# Autodesk Inventor assembly: Baugruppe_Christian_Test
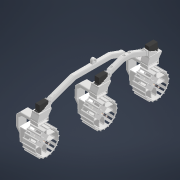
[picture p0: Inventor's stored thumbnail of the model, 180x180]
Saved by Autodesk Inventor 2021 (Build 250183000, 183)
## iProperties
Created: 2021-01-04
Part Number: Baugruppe_Christian_Test
Document SubType Name: Assembly
Designer: Ctroi
Mass: 279.93 g
Surface Area: 1178.31 cm^2
Volume: 279.93 cm^3
Density: 1 g/cm^3
Author: Ctroi
## Documents named in this file (13)
- G:\Roverprojekt\Github Projekt\Rover\Baugruppe_Christian_Test.iam
- G:\Roverprojekt\Github Projekt\Rover\Motorhalterung_v2.ipt
- G:\Roverprojekt\Github Projekt\Rover\Steppermotor.ipt
- G:\Roverprojekt\Github Projekt\Rover\Verbindung_Motor_Servo_v2.ipt
- G:\Roverprojekt\Github Projekt\Rover\Motorhalterung_Klemme.ipt
- G:\Roverprojekt\Github Projekt\Rover\Servohalterung_v2.ipt
- G:\Roverprojekt\Github Projekt\Rover\Servo.ipt
- G:\Roverprojekt\Github Projekt\Rover\Rocker_hinten.ipt
- G:\Roverprojekt\Github Projekt\Rover\Rocker_vorne.ipt
- G:\Roverprojekt\Github Projekt\Rover\Bogie.ipt
- G:\Roverprojekt\Github Projekt\Rover\Servohalterung.ipt
- G:\Roverprojekt\Github Projekt\Rover\Übersetzungsbox_2.ipt
- G:\Roverprojekt\Github Projekt\Rover\Reifen_v2.ipt
## Components (30 placed, 12 different names)
1. Fahrwerk_rocker_hinten:1 — Fluchtend:1, Fluchtend:2, Passend:1, Einfügen:1
2. Fahrwerk_rocker_vorne:1 — Fluchtend:1, Fluchtend:2, Passend:1, Fluchtend:3, Passend:2
3. Fahrwerk_bogie:1 — Einfügen:1, Passend:3, Passend:4
4. Servohalterung:1 — Fluchtend:3, Passend:2, Passend:5
5. Servohalterung:2 — Passend:3, Passend:6, Fluchtend:4
6. Servohalterung:3 — Passend:4, Passend:7, Fluchtend:5, Passend:13
7. Servohalterung_v2:1 — Passend:5, Fluchtend:6, Fluchtend:7, Passend:8, Passend:11
8. Servohalterung_v2:2 — Passend:6, Fluchtend:4, Fluchtend:8, Fluchtend:9, Passend:9, Passend:12
9. Servohalterung_v2:3 — Passend:7, Fluchtend:5, Fluchtend:10, Fluchtend:11, Passend:10
10. Übersetzungsbox_2:1 — Fluchtend:6, Fluchtend:7, Passend:8, Einfügen:2
11. Übersetzungsbox_2:2 — Fluchtend:8, Fluchtend:9, Passend:9, Einfügen:3
12. Übersetzungsbox_2:3 — Fluchtend:10, Fluchtend:11, Passend:10, Einfügen:4
13. Servo:1 — Passend:11
14. Servo:2 — Passend:12
15. Servo:3 — Passend:13
16. Verbindung_Motor_Servo_v2:1 — Einfügen:3, Fluchtend:14, Passend:15, Fluchtend:19
17. Verbindung_Motor_Servo_v2:2 — Einfügen:2, Fluchtend:12, Fluchtend:13, Passend:14
18. Verbindung_Motor_Servo_v2:3 — Einfügen:4, Fluchtend:15, Fluchtend:16, Passend:16
19. Motorhalterung_Klemme:1 — Fluchtend:12, Fluchtend:13, Passend:14, Fluchtend:17, Passend:17, Passend:18
20. Motorhalterung_Klemme:2 — Fluchtend:14, Passend:15, Fluchtend:18, Passend:19, Fluchtend:19, Passend:20
21. Motorhalterung_Klemme:3 — Fluchtend:15, Fluchtend:16, Passend:16, Fluchtend:20, Passend:21, Passend:22
22. Motorhalterung_v2:1 — Fluchtend:17, Passend:17, Passend:18, Passend:23, Passend:24, Passend:25
23. Motorhalterung_v2:2 — Fluchtend:18, Passend:19, Passend:20, Passend:26, Passend:27, Passend:28
24. Motorhalterung_v2:3 — Fluchtend:20, Passend:21, Passend:22, Passend:29, Passend:30, Passend:31
25. Steppermotor:1 — Passend:23, Passend:24, Passend:25, Einfügen:5
26. Steppermotor:2 — Passend:26, Passend:27, Passend:28, Einfügen:6
27. Steppermotor:3 — Passend:29, Passend:30, Passend:31, Einfügen:7
28. Reifen_v2:1 — Einfügen:5
29. Reifen_v2:2 — Einfügen:6
30. Reifen_v2:3 — Einfügen:7
## Relationships (58: Mate 31, Flush 20, Insert 7)
- Fluchtend:1 [Flush]: Fahrwerk_rocker_hinten:1 ↔ Fahrwerk_rocker_vorne:1
- Fluchtend:2 [Flush]: Fahrwerk_rocker_hinten:1 ↔ Fahrwerk_rocker_vorne:1
- Passend:1 [Mate]: Fahrwerk_rocker_hinten:1 ↔ Fahrwerk_rocker_vorne:1
- Einfügen:1 [Insert] (-18 mm): Fahrwerk_rocker_hinten:1 ↔ Fahrwerk_bogie:1
- Fluchtend:3 [Flush]: Fahrwerk_rocker_vorne:1 ↔ Servohalterung:1
- Passend:2 [Mate]: Fahrwerk_rocker_vorne:1 ↔ Servohalterung:1
- Passend:3 [Mate]: Fahrwerk_bogie:1 ↔ Servohalterung:2
- Passend:4 [Mate]: Fahrwerk_bogie:1 ↔ Servohalterung:3
- Passend:5 [Mate]: Servohalterung:1 ↔ Servohalterung_v2:1
- Passend:6 [Mate]: Servohalterung:2 ↔ Servohalterung_v2:2
- Passend:7 [Mate]: Servohalterung:3 ↔ Servohalterung_v2:3
- Fluchtend:4 [Flush] (-2.5 mm): Servohalterung:2 ↔ Servohalterung_v2:2
- Fluchtend:5 [Flush]: Servohalterung:3 ↔ Servohalterung_v2:3
- Fluchtend:6 [Flush]: Servohalterung_v2:1 ↔ Übersetzungsbox_2:1
- Fluchtend:7 [Flush]: Servohalterung_v2:1 ↔ Übersetzungsbox_2:1
- Passend:8 [Mate]: Servohalterung_v2:1 ↔ Übersetzungsbox_2:1
- Fluchtend:8 [Flush]: Servohalterung_v2:2 ↔ Übersetzungsbox_2:2
- Fluchtend:9 [Flush]: Servohalterung_v2:2 ↔ Übersetzungsbox_2:2
- Passend:9 [Mate]: Servohalterung_v2:2 ↔ Übersetzungsbox_2:2
- Fluchtend:10 [Flush]: Servohalterung_v2:3 ↔ Übersetzungsbox_2:3
- Fluchtend:11 [Flush]: Servohalterung_v2:3 ↔ Übersetzungsbox_2:3
- Passend:10 [Mate]: Servohalterung_v2:3 ↔ Übersetzungsbox_2:3
- Passend:11 [Mate]: Servohalterung_v2:1 ↔ Servo:1
- Passend:12 [Mate]: Servohalterung_v2:2 ↔ Servo:2
- Passend:13 [Mate]: Servohalterung:3 ↔ Servo:3
- Einfügen:2 [Insert] (-13 mm): Übersetzungsbox_2:1 ↔ Verbindung_Motor_Servo_v2:2
- Einfügen:3 [Insert] (-13 mm): Übersetzungsbox_2:2 ↔ Verbindung_Motor_Servo_v2:1
- Einfügen:4 [Insert] (-13 mm): Übersetzungsbox_2:3 ↔ Verbindung_Motor_Servo_v2:3
- Fluchtend:12 [Flush]: Verbindung_Motor_Servo_v2:2 ↔ Motorhalterung_Klemme:1
- Fluchtend:13 [Flush]: Verbindung_Motor_Servo_v2:2 ↔ Motorhalterung_Klemme:1
- Passend:14 [Mate]: Verbindung_Motor_Servo_v2:2 ↔ Motorhalterung_Klemme:1
- Fluchtend:14 [Flush]: Verbindung_Motor_Servo_v2:1 ↔ Motorhalterung_Klemme:2
- Passend:15 [Mate]: Verbindung_Motor_Servo_v2:1 ↔ Motorhalterung_Klemme:2
- Fluchtend:15 [Flush]: Verbindung_Motor_Servo_v2:3 ↔ Motorhalterung_Klemme:3
- Fluchtend:16 [Flush]: Verbindung_Motor_Servo_v2:3 ↔ Motorhalterung_Klemme:3
- Passend:16 [Mate]: Verbindung_Motor_Servo_v2:3 ↔ Motorhalterung_Klemme:3
- Fluchtend:17 [Flush]: Motorhalterung_Klemme:1 ↔ Motorhalterung_v2:1
- Passend:17 [Mate]: Motorhalterung_Klemme:1 ↔ Motorhalterung_v2:1
- Passend:18 [Mate]: Motorhalterung_Klemme:1 ↔ Motorhalterung_v2:1
- Fluchtend:18 [Flush]: Motorhalterung_Klemme:2 ↔ Motorhalterung_v2:2
- Passend:19 [Mate]: Motorhalterung_Klemme:2 ↔ Motorhalterung_v2:2
- Fluchtend:19 [Flush]: Verbindung_Motor_Servo_v2:1 ↔ Motorhalterung_Klemme:2
- Passend:20 [Mate]: Motorhalterung_Klemme:2 ↔ Motorhalterung_v2:2
- Fluchtend:20 [Flush]: Motorhalterung_Klemme:3 ↔ Motorhalterung_v2:3
- Passend:21 [Mate]: Motorhalterung_Klemme:3 ↔ Motorhalterung_v2:3
- Passend:22 [Mate]: Motorhalterung_Klemme:3 ↔ Motorhalterung_v2:3
- Passend:23 [Mate]: Motorhalterung_v2:1 ↔ Steppermotor:1
- Passend:24 [Mate]: Motorhalterung_v2:1 ↔ Steppermotor:1
- Passend:25 [Mate]: Motorhalterung_v2:1 ↔ Steppermotor:1
- Passend:26 [Mate]: Motorhalterung_v2:2 ↔ Steppermotor:2
- Passend:27 [Mate]: Motorhalterung_v2:2 ↔ Steppermotor:2
- Passend:28 [Mate]: Motorhalterung_v2:2 ↔ Steppermotor:2
- Passend:29 [Mate]: Motorhalterung_v2:3 ↔ Steppermotor:3
- Passend:30 [Mate]: Motorhalterung_v2:3 ↔ Steppermotor:3
- Passend:31 [Mate]: Motorhalterung_v2:3 ↔ Steppermotor:3
- Einfügen:5 [Insert] (-15 mm): Steppermotor:1 ↔ Reifen_v2:1
- Einfügen:6 [Insert] (-15 mm): Steppermotor:2 ↔ Reifen_v2:2
- Einfügen:7 [Insert] (-15 mm): Steppermotor:3 ↔ Reifen_v2:3
